# Autodesk Inventor assembly: RobotEnvironment
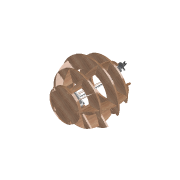
[picture p0: Inventor's stored thumbnail of the model, 180x180]
Saved by Autodesk Inventor 2020.3 (Build 243373000, 373)
## iProperties
Created: 2021-08-02
Part Number: RobotEnvironment
Document SubType Name: Assembly
Designer: justi
Author: justi
## Documents named in this file (3)
- F:\UQ Engineering\2021 ~ 5th Year\Semester 2\METR4911-THESIS\FarmBot CAD\FarmBotV1\RobotEnvironment.iam
- F:\UQ Engineering\2021 ~ 5th Year\Semester 2\METR4911-THESIS\FarmBot CAD\FarmBotV1\FullRobotAssembly.iam
- F:\UQ Engineering\2021 ~ 5th Year\Semester 2\METR4911-THESIS\FarmBot CAD\FarmBotV1\Growroom.iam
## Components (2 placed, 2 different names)
1. FullRobotAssembly:1 [sub-assembly] — Mate:1, Mate:2, Mate:3
2. Growroom:1 [sub-assembly] — Mate:1, Mate:2, Mate:3
## Relationships (3: Mate 3)
- Mate:1: FullRobotAssembly:1 ↔ Growroom:1
- Mate:2: FullRobotAssembly:1 ↔ Growroom:1
- Mate:3: FullRobotAssembly:1 ↔ Growroom:1
